# Autodesk Inventor assembly: Weapon Assembly
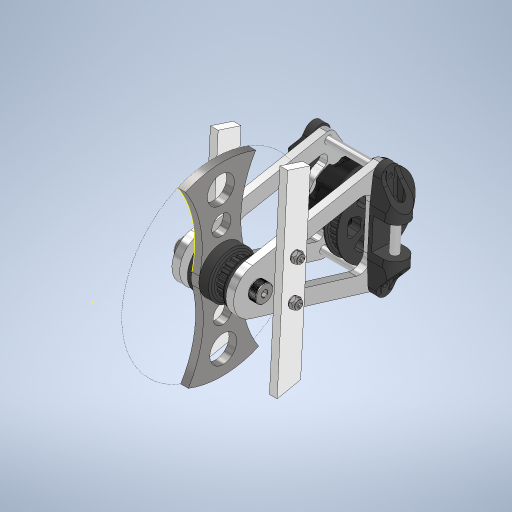
[picture p0: Inventor's stored thumbnail of the model, 512x512]
Saved by Autodesk Inventor 2023.1 (Build 271208000, 208)
## iProperties
Created: 2022-05-21
Part Number: Weapon Assembly
Document SubType Name: Assembly
Designer: Nathan Cai
Mass: 716.023 g
Surface Area: 1380.74 cm^2
Volume: 212.806 cm^3
Density: 3.36467 g/cm^3
Author: Nathan Cai
## Documents named in this file (14)
- E:\Documents\Inventor\0.3rd Lawette - V3.4\Vertical Weapon Assembly\Weapon Assembly.iam
- E:\Documents\Inventor\0.3rd Lawette - V3.4\Vertical Weapon Assembly\Weapon (Weapon-Side Pulley).iam
- E:\Documents\Inventor\0.3rd Lawette - V3.4\Vertical Weapon Assembly\90807A139_Same-Size Thread Alloy Steel Shoulder Screw.ipt
- E:\Documents\Inventor\0.3rd Lawette - V3.4\Vertical Weapon Assembly\90630A121_High-Strength Steel Nylon-Insert Locknut.ipt
- E:\Documents\Inventor\0.3rd Lawette - V3.4\Vertical Weapon Assembly\Weapon (Motor-Side Pulley).iam
- E:\Documents\Inventor\0.3rd Lawette - V3.4\Vertical Weapon Assembly\Frame (Clear Side).ipt
- E:\Documents\Inventor\0.3rd Lawette - V3.4\Standoff 1.5in.ipt
- E:\Documents\Inventor\0.3rd Lawette - V3.4\Vertical Weapon Assembly\Legs.ipt
- E:\Documents\Inventor\Content Center Files\R2023\en-US\ANSI B18.6.3(27)\ANSI B18.6.3 - 6-32 UNC - 0.75(11).ipt
- E:\Documents\Inventor\Content Center Files\R2023\en-US\SAE J773b\SAE J773b - No. 6. SAE Type L. narrow.ipt
- E:\Documents\Inventor\Content Center Files\R2023\en-US\IFI 100 107(2)\IFI 100_107 - No. 6 - 32 Metal Type.ipt
- E:\Documents\Inventor\0.3rd Lawette - V3.4\Vertical Weapon Assembly\Frame (Motor Side).ipt
- E:\Documents\Inventor\0.3rd Lawette - V3.4\Vertical Weapon Assembly\Legs_MIR.ipt
- E:\Documents\Inventor\0.3rd Lawette - V3.4\Bracket.ipt
## Components (26 placed, 13 different names)
1. Weapon (Weapon-Side Pulley):1 [sub-assembly] — Mate:3
2. 90807A139_Same-Size Thread Alloy Steel Shoulder Screw:1 — Mate:1, Mate:2, Mate:3, Mate:9, Mate:10
3. 90630A121_High-Strength Steel Nylon-Insert Locknut:1 — Mate:1, Mate:2
4. Frame (Motor Side):1 — Symmetry:1, Mate:146, Mate:147, Mate:148, Mate:151, Mate:152, Mate:153, Mate:154, Mate:155, Mate:157, Mate:167, Mate:168, Mate:169, Mate:170
5. Frame (Clear Side):1 — Mate:9, Mate:10, Mate:28, Mate:29, Mate:30, Mate:102, Symmetry:1, Mate:159, Mate:160, Mate:161, Mate:162, Mate:163, Mate:165, Mate:173
6. Standoff 1.5in:1 — Mate:102, Mate:171, Mate:174
7. Standoff 1.5in:2 — Mate:172, Mate:175
8. Legs:1 — Mate:28, Mate:29, Mate:30, Mate:164, Mate:166
9. Cross Recessed Truss Head Machine Screw - Type I - Inch No. 6 - 32 - 3/4:8 — Mate:151, Mate:152
10. Conical Spring Washer SAE J773b (Inch) No. 6. SAE Type L. narrow:11 — Mate:155, Mate:156, Insert:21
11. Prevailing Torque Type Hex Nut - Inch (IFI) No. 6 - 32 Metal Type:11 — Insert:21
12. Cross Recessed Truss Head Machine Screw - Type I - Inch No. 6 - 32 - 3/4:10 — Mate:159, Mate:160
13. Conical Spring Washer SAE J773b (Inch) No. 6. SAE Type L. narrow:13 — Mate:163, Mate:164, Insert:23
14. Prevailing Torque Type Hex Nut - Inch (IFI) No. 6 - 32 Metal Type:13 — Insert:23
15. Legs_MIR:1 — Mate:146, Mate:147, Mate:148, Mate:156, Mate:158
16. Cross Recessed Truss Head Machine Screw - Type I - Inch No. 6 - 32 - 3/4:14 — Mate:153, Mate:154
17. Conical Spring Washer SAE J773b (Inch) No. 6. SAE Type L. narrow:17 — Mate:157, Mate:158, Insert:22
18. Prevailing Torque Type Hex Nut - Inch (IFI) No. 6 - 32 Metal Type:17 — Insert:22
19. Cross Recessed Truss Head Machine Screw - Type I - Inch No. 6 - 32 - 3/4:15 — Mate:161, Mate:162
20. Conical Spring Washer SAE J773b (Inch) No. 6. SAE Type L. narrow:18 — Mate:165, Mate:166, Insert:24
21. Prevailing Torque Type Hex Nut - Inch (IFI) No. 6 - 32 Metal Type:18 — Insert:24
22. Weapon (Motor-Side Pulley):1 [sub-assembly] — Mate:167, Mate:168, Mate:169
23. Bracket:1 — Mate:173, Mate:174, Mate:175, Mate:176, Flush:2
24. Bracket:2 — Mate:170, Mate:171, Mate:172, Mate:177, Flush:1
25. Standoff 1.5in:3 — Mate:176, Flush:2
26. Standoff 1.5in:4 — Mate:177, Flush:1
## Relationships (53: Mate 46, Insert 4, Flush 2, Symmetry 1)
- Mate:1: 90807A139_Same-Size Thread Alloy Steel Shoulder Screw:1 ↔ 90630A121_High-Strength Steel Nylon-Insert Locknut:1
- Mate:2 (50.8 mm): 90807A139_Same-Size Thread Alloy Steel Shoulder Screw:1 ↔ 90630A121_High-Strength Steel Nylon-Insert Locknut:1
- Mate:3: Weapon (Weapon-Side Pulley):1 ↔ 90807A139_Same-Size Thread Alloy Steel Shoulder Screw:1
- [Mate]: 90807A139_Same-Size Thread Alloy Steel Shoulder Screw:1 ↔ Frame (Motor Side):1
- Mate:9: 90807A139_Same-Size Thread Alloy Steel Shoulder Screw:1 ↔ Frame (Clear Side):1
- Mate:10: 90807A139_Same-Size Thread Alloy Steel Shoulder Screw:1 ↔ Frame (Clear Side):1
- [Mate]: Frame (Motor Side):1 ↔ Frame (Clear Side):1
- [Mate]: Frame (Motor Side):1 ↔ Standoff 1.5in:1
- [Mate]: Frame (Motor Side):1 ↔ Standoff 1.5in:2
- [Mate]: Frame (Motor Side):1 ↔ Standoff 1.5in:1
- [Mate]: Frame (Motor Side):1 ↔ Standoff 1.5in:2
- Mate:28: Frame (Clear Side):1 ↔ Legs:1
- Mate:29: Frame (Clear Side):1 ↔ Legs:1
- Mate:30: Frame (Clear Side):1 ↔ Legs:1
- Mate:102: Frame (Clear Side):1 ↔ Standoff 1.5in:1
- [Mate] (0.0254 mm): Weapon (Weapon-Side Pulley):1 ↔ Frame (Motor Side):1
- Symmetry:1: Frame (Motor Side):1 ↔ Frame (Clear Side):1
- Mate:146: Frame (Motor Side):1 ↔ Legs_MIR:1
- Mate:147: Frame (Motor Side):1 ↔ Legs_MIR:1
- Mate:148: Frame (Motor Side):1 ↔ Legs_MIR:1
- Mate:151: Frame (Motor Side):1 ↔ Cross Recessed Truss Head Machine Screw - Type I - Inch No. 6 - 32 - 3/4:8
- Mate:152: Frame (Motor Side):1 ↔ Cross Recessed Truss Head Machine Screw - Type I - Inch No. 6 - 32 - 3/4:8
- Mate:153: Frame (Motor Side):1 ↔ Cross Recessed Truss Head Machine Screw - Type I - Inch No. 6 - 32 - 3/4:14
- Mate:154: Frame (Motor Side):1 ↔ Cross Recessed Truss Head Machine Screw - Type I - Inch No. 6 - 32 - 3/4:14
- Mate:155: Frame (Motor Side):1 ↔ Conical Spring Washer SAE J773b (Inch) No. 6. SAE Type L. narrow:11
- Mate:156: Conical Spring Washer SAE J773b (Inch) No. 6. SAE Type L. narrow:11 ↔ Legs_MIR:1
- Mate:157: Frame (Motor Side):1 ↔ Conical Spring Washer SAE J773b (Inch) No. 6. SAE Type L. narrow:17
- Mate:158: Legs_MIR:1 ↔ Conical Spring Washer SAE J773b (Inch) No. 6. SAE Type L. narrow:17
- Insert:21: Conical Spring Washer SAE J773b (Inch) No. 6. SAE Type L. narrow:11 ↔ Prevailing Torque Type Hex Nut - Inch (IFI) No. 6 - 32 Metal Type:11
- Insert:22: Conical Spring Washer SAE J773b (Inch) No. 6. SAE Type L. narrow:17 ↔ Prevailing Torque Type Hex Nut - Inch (IFI) No. 6 - 32 Metal Type:17
- Mate:159: Frame (Clear Side):1 ↔ Cross Recessed Truss Head Machine Screw - Type I - Inch No. 6 - 32 - 3/4:10
- Mate:160: Frame (Clear Side):1 ↔ Cross Recessed Truss Head Machine Screw - Type I - Inch No. 6 - 32 - 3/4:10
- Mate:161: Frame (Clear Side):1 ↔ Cross Recessed Truss Head Machine Screw - Type I - Inch No. 6 - 32 - 3/4:15
- Mate:162: Frame (Clear Side):1 ↔ Cross Recessed Truss Head Machine Screw - Type I - Inch No. 6 - 32 - 3/4:15
- Mate:163: Frame (Clear Side):1 ↔ Conical Spring Washer SAE J773b (Inch) No. 6. SAE Type L. narrow:13
- Mate:164: Legs:1 ↔ Conical Spring Washer SAE J773b (Inch) No. 6. SAE Type L. narrow:13
- Mate:165: Frame (Clear Side):1 ↔ Conical Spring Washer SAE J773b (Inch) No. 6. SAE Type L. narrow:18
- Mate:166: Legs:1 ↔ Conical Spring Washer SAE J773b (Inch) No. 6. SAE Type L. narrow:18
- Insert:23: Conical Spring Washer SAE J773b (Inch) No. 6. SAE Type L. narrow:13 ↔ Prevailing Torque Type Hex Nut - Inch (IFI) No. 6 - 32 Metal Type:13
- Insert:24: Conical Spring Washer SAE J773b (Inch) No. 6. SAE Type L. narrow:18 ↔ Prevailing Torque Type Hex Nut - Inch (IFI) No. 6 - 32 Metal Type:18
- Mate:167: Frame (Motor Side):1 ↔ Weapon (Motor-Side Pulley):1
- Mate:168: Frame (Motor Side):1 ↔ Weapon (Motor-Side Pulley):1
- Mate:169: Frame (Motor Side):1 ↔ Weapon (Motor-Side Pulley):1
- Mate:170: Frame (Motor Side):1 ↔ Bracket:2
- Mate:171: Standoff 1.5in:1 ↔ Bracket:2
- Mate:172: Standoff 1.5in:2 ↔ Bracket:2
- Mate:173: Frame (Clear Side):1 ↔ Bracket:1
- Mate:174: Standoff 1.5in:1 ↔ Bracket:1
- Mate:175: Standoff 1.5in:2 ↔ Bracket:1
- Mate:176: Bracket:1 ↔ Standoff 1.5in:3
- Mate:177: Bracket:2 ↔ Standoff 1.5in:4
- Flush:1: Bracket:2 ↔ Standoff 1.5in:4
- Flush:2: Bracket:1 ↔ Standoff 1.5in:3
